# Autodesk Inventor assembly: bevel gear + hyper hub 8mm rex
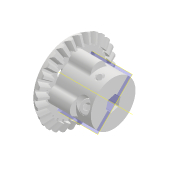
[picture p0: Inventor's stored thumbnail of the model, 180x180]
Saved by Autodesk Inventor 2020 (Build 240168000, 168)
## iProperties
Created: 2020-02-26
Part Number: bevel gear + hyper hub 8mm rex
Document SubType Name: Assembly
Designer: ball
Author: ball
## Documents named in this file (4)
- C:\FTC\FTC8863CAD\2019 Robot\Mecanum Drive Train Metal\bevel gear + hyper hub 8mm rex.iam
- C:\FTC\FTC8863CAD\GoBilda\2307 parts\2307-0014-0028.ipt
- C:\FTC\FTC8863CAD\GoBilda\1310 Parts\1310-0016-4008 assembly.ipt
- C:\FTC\FTC8863CAD\StepLibraries\Screws\M4 x 12 SOCKET HEAD CAP SCREW.ipt
## Components (6 placed, 3 different names)
1. 2307-0014-0028:1 — Mate:1, Mate:2, Mate:3, Mate:4, Mate:5, Mate:7, Mate:9, Mate:11
2. 1310-0016-4008 assembly:1 — Mate:1, Mate:2, Mate:3, Mate:4, Mate:6, Mate:8, Mate:10, Mate:12, Mate:13
3. M4 x 12 SOCKET HEAD CAP SCREW:1 — Mate:5, Mate:6
4. M4 x 12 SOCKET HEAD CAP SCREW:2 — Mate:9, Mate:10
5. M4 x 12 SOCKET HEAD CAP SCREW:3 — Mate:11, Mate:12, Mate:13
6. M4 x 12 SOCKET HEAD CAP SCREW:4 — Mate:7, Mate:8
## Relationships (13: Mate 13)
- Mate:1: 2307-0014-0028:1 ↔ 1310-0016-4008 assembly:1
- Mate:2: 2307-0014-0028:1 ↔ 1310-0016-4008 assembly:1
- Mate:3: 2307-0014-0028:1 ↔ 1310-0016-4008 assembly:1
- Mate:4: 2307-0014-0028:1 ↔ 1310-0016-4008 assembly:1
- Mate:5: 2307-0014-0028:1 ↔ M4 x 12 SOCKET HEAD CAP SCREW:1
- Mate:6: 1310-0016-4008 assembly:1 ↔ M4 x 12 SOCKET HEAD CAP SCREW:1
- Mate:7: 2307-0014-0028:1 ↔ M4 x 12 SOCKET HEAD CAP SCREW:4
- Mate:8: 1310-0016-4008 assembly:1 ↔ M4 x 12 SOCKET HEAD CAP SCREW:4
- Mate:9: 2307-0014-0028:1 ↔ M4 x 12 SOCKET HEAD CAP SCREW:2
- Mate:10: 1310-0016-4008 assembly:1 ↔ M4 x 12 SOCKET HEAD CAP SCREW:2
- Mate:11: 2307-0014-0028:1 ↔ M4 x 12 SOCKET HEAD CAP SCREW:3
- Mate:12: 1310-0016-4008 assembly:1 ↔ M4 x 12 SOCKET HEAD CAP SCREW:3
- Mate:13: 1310-0016-4008 assembly:1 ↔ M4 x 12 SOCKET HEAD CAP SCREW:3
